# Autodesk Inventor assembly: NXT Asem
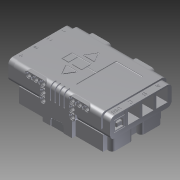
[picture p0: Inventor's stored thumbnail of the model, 180x180]
Saved by Autodesk Inventor 2012 (Build 160160000, 160)
## iProperties
Created: 2011-01-03
Part Number: NXT Asem
Document SubType Name: Assembly
Designer: AndrewRemmers
Author: AndrewRemmers
## Documents named in this file (3)
- C:\Users\Andrew\Documents\Inventor\FTC 2010 GET OVER IT\FTC CAD Database\FTC CAD Files\Electrical\NXT Asem.iam
- C:\Users\Andrew\Documents\Inventor\FTC 2010 GET OVER IT\Imported Components\nxt_battery_door\nxt_battery_door.ipt
- C:\Users\Andrew\Documents\Inventor\FTC 2010 GET OVER IT\Imported Components\nxt2\nxt2.ipt
## Components (2 placed, 2 different names)
1. nxt_battery_door:1 — Mate:1, Mate:2, Mate:3
2. nxt2:1 — Mate:1, Mate:2, Mate:3
## Relationships (3: Mate 3)
- Mate:1: nxt_battery_door:1 ↔ nxt2:1
- Mate:2: nxt_battery_door:1 ↔ nxt2:1
- Mate:3: nxt_battery_door:1 ↔ nxt2:1
